# Autodesk Inventor assembly: kadlub_assembly
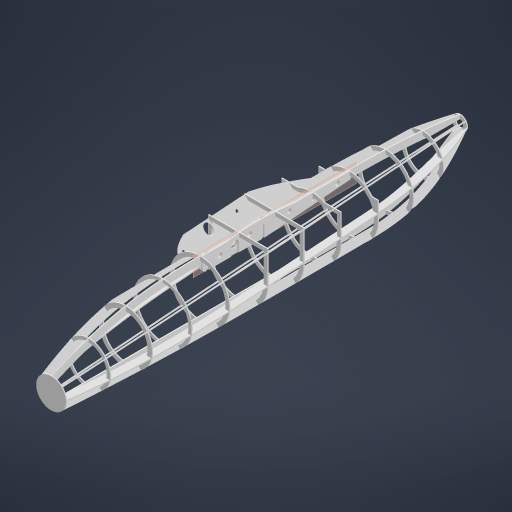
[picture p0: Inventor's stored thumbnail of the model, 512x512]
Saved by Autodesk Inventor 2023 (Build 270158000, 158)
## iProperties
Created: 2023-01-02
Part Number: kadlub_assembly
Document SubType Name: Assembly
Designer: Maciej
Author: Maciej
## Documents named in this file (23)
- D:\Folder Instalacyjny\GitHub Pliki\Solaris\new model\kadlub_assembly.iam
- D:\Folder Instalacyjny\GitHub Pliki\Solaris\new model\Part1.ipt
- D:\Folder Instalacyjny\GitHub Pliki\Solaris\new model\Part2.ipt
- D:\Folder Instalacyjny\GitHub Pliki\Solaris\new model\Part3.ipt
- D:\Folder Instalacyjny\GitHub Pliki\Solaris\new model\Part4.ipt
- D:\Folder Instalacyjny\GitHub Pliki\Solaris\new model\Part5.ipt
- D:\Folder Instalacyjny\GitHub Pliki\Solaris\new model\Part6.ipt
- D:\Folder Instalacyjny\GitHub Pliki\Solaris\new model\Part7.ipt
- D:\Folder Instalacyjny\GitHub Pliki\Solaris\new model\Part8.ipt
- D:\Folder Instalacyjny\GitHub Pliki\Solaris\new model\Part9.ipt
- D:\Folder Instalacyjny\GitHub Pliki\Solaris\new model\Part10.ipt
- D:\Folder Instalacyjny\GitHub Pliki\Solaris\new model\Part11.ipt
- D:\Folder Instalacyjny\GitHub Pliki\Solaris\new model\Part12.ipt
- D:\Folder Instalacyjny\GitHub Pliki\Solaris\new model\Part13.ipt
- D:\Folder Instalacyjny\GitHub Pliki\Solaris\new model\Part14.ipt
- D:\Folder Instalacyjny\GitHub Pliki\Solaris\new model\Part15.ipt
- D:\Folder Instalacyjny\GitHub Pliki\Solaris\new model\Part16.ipt
- D:\Folder Instalacyjny\GitHub Pliki\Solaris\new model\Part17.ipt
- D:\Folder Instalacyjny\GitHub Pliki\Solaris\new model\Part18.ipt
- D:\Folder Instalacyjny\GitHub Pliki\Solaris\new model\Part19.ipt
- D:\Folder Instalacyjny\GitHub Pliki\Solaris\new model\Part20.ipt
- D:\Folder Instalacyjny\GitHub Pliki\Solaris\new model\Part21.ipt
- D:\Folder Instalacyjny\GitHub Pliki\Solaris\new model\Part22.ipt
## Components (22 placed, 22 different names)
1. Part1:1
2. Part2:1
3. Part3:1
4. Part4:1
5. Part5:1
6. Part6:1
7. Part7:1
8. Part8:1
9. Part9:1
10. Part10:1
11. Part11:1
12. Part12:1
13. Part13:1 — Flush:4
14. Part14:1
15. Part15:1
16. Part16:1
17. Part17:1 — Flush:5
18. Part18:1
19. Part19:1 — Flush:1, Flush:4
20. Part20:1
21. Part21:1 — Flush:5, Symmetry:1
22. Part22:1 — Flush:1, Symmetry:1
## Relationships (4: Flush 3, Symmetry 1)
- Flush:1: Part19:1 ↔ Part22:1
- Flush:4: Part13:1 ↔ Part19:1
- Flush:5: Part17:1 ↔ Part21:1
- Symmetry:1: Part21:1 ↔ Part22:1
